# Autodesk Inventor assembly: GI - 100
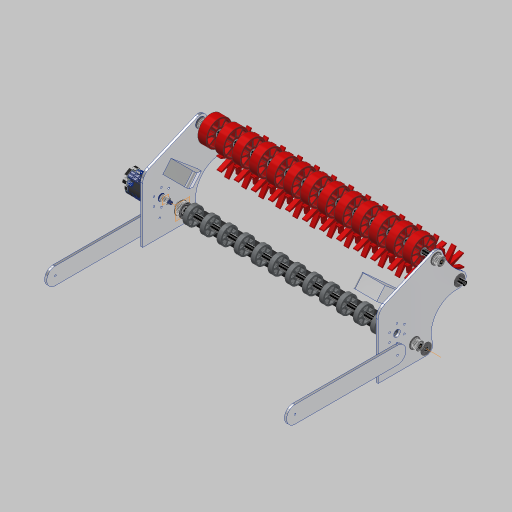
[picture p0: Inventor's stored thumbnail of the model, 512x512]
Saved by Autodesk Inventor 2023.5 (Build 275446000, 446)
## iProperties
Created: 2025-01-18
Part Number: GI - 100
Document SubType Name: Assembly
Designer: mavericks
Author: mavericks
## Documents named in this file (14)
- C:\Users\slick\OneDrive\Desktop\2025-ReefScape---CAD\ground intake\GI - 100.iam
- C:\Users\slick\OneDrive\Desktop\2025-ReefScape---CAD\ground intake\GI - 001.ipt
- C:\Users\slick\OneDrive\Desktop\2025-ReefScape---CAD\COMMON PARTS\BEARINGS\13_75mm_1_2_ThunderHex_ID_x_1_125_OD_x_0_313_WD_Flanged_Bearing_217-4006_MIR.ipt
- C:\Users\slick\OneDrive\Desktop\2025-ReefScape---CAD\ground intake\GI - 002.ipt
- C:\Users\slick\OneDrive\Desktop\2025-ReefScape---CAD\COMMON PARTS\WHEELS\am-0619a .425 Hex Entrapption Star REV2.ipt
- C:\Users\slick\OneDrive\Desktop\2025-ReefScape---CAD\COMMON PARTS\WHEELS\am-3946 3IN 375Hex Compliant Wheel REV 3.ipt
- C:\Users\slick\OneDrive\Desktop\2025-ReefScape---CAD\COMMON PARTS\WHEELS\2_OD_Straight_Flex_Wheel_217-6354.ipt
- C:\Users\slick\OneDrive\Desktop\2025-ReefScape---CAD\ground intake\GI - 200.iam
- C:\Users\slick\OneDrive\Desktop\2025-ReefScape---CAD\COMMON PARTS\MOTORS\Kracken with Cover and Boards.iam
- C:\Users\slick\OneDrive\Desktop\2025-ReefScape---CAD\COMMON PARTS\PULLEYS\gt2\16T Gt2 Kracken PullyWCP-1178.ipt
- C:\Users\slick\OneDrive\Desktop\2025-ReefScape---CAD\COMMON PARTS\PULLEYS\gt2\24t_x_9mm_Wide_Double_Flange_Aluminum_Pulley_GT2_3mm_1_2_Hex_Bore_217-5875.ipt
- C:\Users\slick\OneDrive\Desktop\2025-ReefScape---CAD\COMMON PARTS\PULLEYS\gt2\36t_x_9mm_Wide_Double_Flange_Aluminum_Pulley_GT2_3mm_1_2_Hex_Bore_217-5873.ipt
- C:\Users\slick\OneDrive\Desktop\2025-ReefScape---CAD\ground intake\GI - 005.ipt
- C:\Users\slick\OneDrive\Desktop\2025-ReefScape---CAD\ground intake\GI - 006.ipt
## Components (66 placed, 13 different names)
1. GI - 001:1 — Insert:1, Insert:2, Insert:3, Insert:4, Mate:2, Mate:4, Mate:6, Insert:18, Mate:7, Mate:15, Mate:28, Angle:1, Mate:30, Insert:21
2. 13_75mm_1_2_ThunderHex_ID_x_1_125_OD_x_0_313_WD_Flanged_Bearing_217-4006_MIR:1 — Insert:2, Mate:1, Flush:2, Mate:15, Mate:16, Flush:5, Mate:25, Mate:26
3. 13_75mm_1_2_ThunderHex_ID_x_1_125_OD_x_0_313_WD_Flanged_Bearing_217-4006_MIR:2 — Insert:1, Mate:3, Flush:4, Mate:23, Mate:24
4. 13_75mm_1_2_ThunderHex_ID_x_1_125_OD_x_0_313_WD_Flanged_Bearing_217-4006_MIR:3 — Insert:4, Insert:19
5. 13_75mm_1_2_ThunderHex_ID_x_1_125_OD_x_0_313_WD_Flanged_Bearing_217-4006_MIR:4 — Insert:3, Mate:5, Mate:10, Mate:11, Mate:12, Mate:20, Mate:21
6. GI - 001:2 — Insert:5, Insert:6, Insert:7, Insert:8, Mate:29, Mate:31, Insert:20, Angle:2
7. 13_75mm_1_2_ThunderHex_ID_x_1_125_OD_x_0_313_WD_Flanged_Bearing_217-4006_MIR:5 — Insert:5, Mate:19
8. 13_75mm_1_2_ThunderHex_ID_x_1_125_OD_x_0_313_WD_Flanged_Bearing_217-4006_MIR:6 — Insert:6, Mate:18
9. 13_75mm_1_2_ThunderHex_ID_x_1_125_OD_x_0_313_WD_Flanged_Bearing_217-4006_MIR:7 — Insert:8, Insert:16, Mate:14
10. 13_75mm_1_2_ThunderHex_ID_x_1_125_OD_x_0_313_WD_Flanged_Bearing_217-4006_MIR:8 — Insert:7
11. GI - 002:1 — Mate:18, Flush:4, Mate:27
12. GI - 002:2 — Mate:17, Flush:3, Mate:20, Mate:21
13. GI - 002:4 — Flush:2, Mate:16, Mate:19, Flush:5, Flush:6
14. GI - 200:1 [sub-assembly] — Insert:16, Mate:13, Insert:19
15. Kracken with Cover and Boards:1 [sub-assembly] — Insert:18, Mate:7, Mate:8, Mate:9, Mate:32
16. 16T Gt2 Kracken PullyWCP-1178:1 — Mate:8, Mate:9
17. 24t_x_9mm_Wide_Double_Flange_Aluminum_Pulley_GT2_3mm_1_2_Hex_Bore_217-5875:1 — Mate:10, Flush:1
18. 36t_x_9mm_Wide_Double_Flange_Aluminum_Pulley_GT2_3mm_1_2_Hex_Bore_217-5873:1 — Mate:11, Mate:12
19. 24t_x_9mm_Wide_Double_Flange_Aluminum_Pulley_GT2_3mm_1_2_Hex_Bore_217-5875:2 — Mate:13, Mate:14, Flush:1
20. 24t_x_9mm_Wide_Double_Flange_Aluminum_Pulley_GT2_3mm_1_2_Hex_Bore_217-5875:3 — Mate:17, Flush:3
21. 24t_x_9mm_Wide_Double_Flange_Aluminum_Pulley_GT2_3mm_1_2_Hex_Bore_217-5875:4 — Flush:6, Mate:27
22. 24t_x_9mm_Wide_Double_Flange_Aluminum_Pulley_GT2_3mm_1_2_Hex_Bore_217-5875:5 — Mate:23, Mate:24
23. 24t_x_9mm_Wide_Double_Flange_Aluminum_Pulley_GT2_3mm_1_2_Hex_Bore_217-5875:6 — Mate:25, Mate:26
24. GI - 005:1 — Mate:28, Flush:7, Angle:1, Mate:30, Mate:32
25. GI - 005:2 — Mate:29, Flush:7, Mate:31
26. GI - 006:1 — Insert:20, Angle:2, Flush:8
27. GI - 006:2 — Insert:21, Flush:8
28. am-0619a .425 Hex Entrapption Star REV2:1 — Mate:1, Mate:2
29. am-0619a .425 Hex Entrapption Star REV2:2
30. am-0619a .425 Hex Entrapption Star REV2:3
31. am-0619a .425 Hex Entrapption Star REV2:4
32. am-0619a .425 Hex Entrapption Star REV2:5
33. am-0619a .425 Hex Entrapption Star REV2:6
34. am-0619a .425 Hex Entrapption Star REV2:7
35. am-0619a .425 Hex Entrapption Star REV2:8
36. am-0619a .425 Hex Entrapption Star REV2:9
37. am-0619a .425 Hex Entrapption Star REV2:10
38. am-0619a .425 Hex Entrapption Star REV2:11
39. am-0619a .425 Hex Entrapption Star REV2:12
40. am-0619a .425 Hex Entrapption Star REV2:13
41. am-3946 3IN 375Hex Compliant Wheel REV 3:1 — Mate:3, Mate:4
42. am-3946 3IN 375Hex Compliant Wheel REV 3:2
43. am-3946 3IN 375Hex Compliant Wheel REV 3:3
44. am-3946 3IN 375Hex Compliant Wheel REV 3:4
45. am-3946 3IN 375Hex Compliant Wheel REV 3:5
46. am-3946 3IN 375Hex Compliant Wheel REV 3:6
47. am-3946 3IN 375Hex Compliant Wheel REV 3:7
48. am-3946 3IN 375Hex Compliant Wheel REV 3:8
49. am-3946 3IN 375Hex Compliant Wheel REV 3:9
50. am-3946 3IN 375Hex Compliant Wheel REV 3:10
51. am-3946 3IN 375Hex Compliant Wheel REV 3:11
52. am-3946 3IN 375Hex Compliant Wheel REV 3:12
53. am-3946 3IN 375Hex Compliant Wheel REV 3:13
54. 2_OD_Straight_Flex_Wheel_217-6354:1 — Mate:5, Mate:6
55. 2_OD_Straight_Flex_Wheel_217-6354:2
56. 2_OD_Straight_Flex_Wheel_217-6354:3
57. 2_OD_Straight_Flex_Wheel_217-6354:4
58. 2_OD_Straight_Flex_Wheel_217-6354:5
59. 2_OD_Straight_Flex_Wheel_217-6354:6
60. 2_OD_Straight_Flex_Wheel_217-6354:7
61. 2_OD_Straight_Flex_Wheel_217-6354:8
62. 2_OD_Straight_Flex_Wheel_217-6354:9
63. 2_OD_Straight_Flex_Wheel_217-6354:10
64. 2_OD_Straight_Flex_Wheel_217-6354:11
65. 2_OD_Straight_Flex_Wheel_217-6354:12
66. 2_OD_Straight_Flex_Wheel_217-6354:13
## Component patterns: (13 elements, first: am-0619a .425 Hex Entrapption Star REV2:1), (13 elements, first: am-3946 3IN 375Hex Compliant Wheel REV 3:1), (13 elements, first: 2_OD_Straight_Flex_Wheel_217-6354:1)
## Relationships (54: Mate 31, Insert 13, Flush 8, Angle 2)
- Insert:1: GI - 001:1 ↔ 13_75mm_1_2_ThunderHex_ID_x_1_125_OD_x_0_313_WD_Flanged_Bearing_217-4006_MIR:2
- Insert:2: GI - 001:1 ↔ 13_75mm_1_2_ThunderHex_ID_x_1_125_OD_x_0_313_WD_Flanged_Bearing_217-4006_MIR:1
- Insert:3: GI - 001:1 ↔ 13_75mm_1_2_ThunderHex_ID_x_1_125_OD_x_0_313_WD_Flanged_Bearing_217-4006_MIR:4
- Insert:4: GI - 001:1 ↔ 13_75mm_1_2_ThunderHex_ID_x_1_125_OD_x_0_313_WD_Flanged_Bearing_217-4006_MIR:3
- Insert:5: GI - 001:2 ↔ 13_75mm_1_2_ThunderHex_ID_x_1_125_OD_x_0_313_WD_Flanged_Bearing_217-4006_MIR:5
- Insert:6: GI - 001:2 ↔ 13_75mm_1_2_ThunderHex_ID_x_1_125_OD_x_0_313_WD_Flanged_Bearing_217-4006_MIR:6
- Insert:7: GI - 001:2 ↔ 13_75mm_1_2_ThunderHex_ID_x_1_125_OD_x_0_313_WD_Flanged_Bearing_217-4006_MIR:8
- Insert:8: GI - 001:2 ↔ 13_75mm_1_2_ThunderHex_ID_x_1_125_OD_x_0_313_WD_Flanged_Bearing_217-4006_MIR:7
- Mate:1: 13_75mm_1_2_ThunderHex_ID_x_1_125_OD_x_0_313_WD_Flanged_Bearing_217-4006_MIR:1 ↔ am-0619a .425 Hex Entrapption Star REV2:1
- Mate:2 (36.5125 mm): GI - 001:1 ↔ am-0619a .425 Hex Entrapption Star REV2:1
- Mate:3: 13_75mm_1_2_ThunderHex_ID_x_1_125_OD_x_0_313_WD_Flanged_Bearing_217-4006_MIR:2 ↔ am-3946 3IN 375Hex Compliant Wheel REV 3:1
- Mate:4 (30.1625 mm): GI - 001:1 ↔ am-3946 3IN 375Hex Compliant Wheel REV 3:1
- Mate:5: 13_75mm_1_2_ThunderHex_ID_x_1_125_OD_x_0_313_WD_Flanged_Bearing_217-4006_MIR:4 ↔ 2_OD_Straight_Flex_Wheel_217-6354:1
- Mate:6 (36.5125 mm): GI - 001:1 ↔ 2_OD_Straight_Flex_Wheel_217-6354:1
- Insert:16: 13_75mm_1_2_ThunderHex_ID_x_1_125_OD_x_0_313_WD_Flanged_Bearing_217-4006_MIR:7 ↔ GI - 200:1
- Insert:18: GI - 001:1 ↔ Kracken with Cover and Boards:1
- Mate:7: GI - 001:1 ↔ Kracken with Cover and Boards:1
- Mate:8: Kracken with Cover and Boards:1 ↔ 16T Gt2 Kracken PullyWCP-1178:1
- Mate:9 (3.175 mm): Kracken with Cover and Boards:1 ↔ 16T Gt2 Kracken PullyWCP-1178:1
- Mate:10: 13_75mm_1_2_ThunderHex_ID_x_1_125_OD_x_0_313_WD_Flanged_Bearing_217-4006_MIR:4 ↔ 24t_x_9mm_Wide_Double_Flange_Aluminum_Pulley_GT2_3mm_1_2_Hex_Bore_217-5875:1
- Mate:11: 13_75mm_1_2_ThunderHex_ID_x_1_125_OD_x_0_313_WD_Flanged_Bearing_217-4006_MIR:4 ↔ 36t_x_9mm_Wide_Double_Flange_Aluminum_Pulley_GT2_3mm_1_2_Hex_Bore_217-5873:1
- Mate:12 (3.175 mm): 13_75mm_1_2_ThunderHex_ID_x_1_125_OD_x_0_313_WD_Flanged_Bearing_217-4006_MIR:4 ↔ 36t_x_9mm_Wide_Double_Flange_Aluminum_Pulley_GT2_3mm_1_2_Hex_Bore_217-5873:1
- Mate:13: GI - 200:1 ↔ 24t_x_9mm_Wide_Double_Flange_Aluminum_Pulley_GT2_3mm_1_2_Hex_Bore_217-5875:2
- Mate:14: 13_75mm_1_2_ThunderHex_ID_x_1_125_OD_x_0_313_WD_Flanged_Bearing_217-4006_MIR:7 ↔ 24t_x_9mm_Wide_Double_Flange_Aluminum_Pulley_GT2_3mm_1_2_Hex_Bore_217-5875:2
- Flush:1: 24t_x_9mm_Wide_Double_Flange_Aluminum_Pulley_GT2_3mm_1_2_Hex_Bore_217-5875:1 ↔ 24t_x_9mm_Wide_Double_Flange_Aluminum_Pulley_GT2_3mm_1_2_Hex_Bore_217-5875:2
- Flush:2: 13_75mm_1_2_ThunderHex_ID_x_1_125_OD_x_0_313_WD_Flanged_Bearing_217-4006_MIR:1 ↔ GI - 002:4
- Mate:15: GI - 001:1 ↔ 13_75mm_1_2_ThunderHex_ID_x_1_125_OD_x_0_313_WD_Flanged_Bearing_217-4006_MIR:1
- Mate:16: 13_75mm_1_2_ThunderHex_ID_x_1_125_OD_x_0_313_WD_Flanged_Bearing_217-4006_MIR:1 ↔ GI - 002:4
- Insert:19: 13_75mm_1_2_ThunderHex_ID_x_1_125_OD_x_0_313_WD_Flanged_Bearing_217-4006_MIR:3 ↔ GI - 200:1
- Mate:17: GI - 002:2 ↔ 24t_x_9mm_Wide_Double_Flange_Aluminum_Pulley_GT2_3mm_1_2_Hex_Bore_217-5875:3
- Flush:3: GI - 002:2 ↔ 24t_x_9mm_Wide_Double_Flange_Aluminum_Pulley_GT2_3mm_1_2_Hex_Bore_217-5875:3
- Mate:18: 13_75mm_1_2_ThunderHex_ID_x_1_125_OD_x_0_313_WD_Flanged_Bearing_217-4006_MIR:6 ↔ GI - 002:1
- Mate:19: 13_75mm_1_2_ThunderHex_ID_x_1_125_OD_x_0_313_WD_Flanged_Bearing_217-4006_MIR:5 ↔ GI - 002:4
- Flush:4: 13_75mm_1_2_ThunderHex_ID_x_1_125_OD_x_0_313_WD_Flanged_Bearing_217-4006_MIR:2 ↔ GI - 002:1
- Flush:5: 13_75mm_1_2_ThunderHex_ID_x_1_125_OD_x_0_313_WD_Flanged_Bearing_217-4006_MIR:1 ↔ GI - 002:4
- Mate:20: 13_75mm_1_2_ThunderHex_ID_x_1_125_OD_x_0_313_WD_Flanged_Bearing_217-4006_MIR:4 ↔ GI - 002:2
- Mate:21: 13_75mm_1_2_ThunderHex_ID_x_1_125_OD_x_0_313_WD_Flanged_Bearing_217-4006_MIR:4 ↔ GI - 002:2
- Flush:6: GI - 002:4 ↔ 24t_x_9mm_Wide_Double_Flange_Aluminum_Pulley_GT2_3mm_1_2_Hex_Bore_217-5875:4
- Mate:23: 13_75mm_1_2_ThunderHex_ID_x_1_125_OD_x_0_313_WD_Flanged_Bearing_217-4006_MIR:2 ↔ 24t_x_9mm_Wide_Double_Flange_Aluminum_Pulley_GT2_3mm_1_2_Hex_Bore_217-5875:5
- Mate:24 (3.175 mm): 13_75mm_1_2_ThunderHex_ID_x_1_125_OD_x_0_313_WD_Flanged_Bearing_217-4006_MIR:2 ↔ 24t_x_9mm_Wide_Double_Flange_Aluminum_Pulley_GT2_3mm_1_2_Hex_Bore_217-5875:5
- Mate:25: 13_75mm_1_2_ThunderHex_ID_x_1_125_OD_x_0_313_WD_Flanged_Bearing_217-4006_MIR:1 ↔ 24t_x_9mm_Wide_Double_Flange_Aluminum_Pulley_GT2_3mm_1_2_Hex_Bore_217-5875:6
- Mate:26 (3.175 mm): 13_75mm_1_2_ThunderHex_ID_x_1_125_OD_x_0_313_WD_Flanged_Bearing_217-4006_MIR:1 ↔ 24t_x_9mm_Wide_Double_Flange_Aluminum_Pulley_GT2_3mm_1_2_Hex_Bore_217-5875:6
- Mate:27: GI - 002:1 ↔ 24t_x_9mm_Wide_Double_Flange_Aluminum_Pulley_GT2_3mm_1_2_Hex_Bore_217-5875:4
- Mate:28: GI - 001:1 ↔ GI - 005:1
- Mate:29: GI - 001:2 ↔ GI - 005:2
- Flush:7: GI - 005:1 ↔ GI - 005:2
- Angle:1 (40 deg): GI - 001:1 ↔ GI - 005:1
- Mate:30 (101.6 mm): GI - 001:1 ↔ GI - 005:1
- Mate:31 (177.8 mm): GI - 001:2 ↔ GI - 005:2
- Mate:32 (57.15 mm): Kracken with Cover and Boards:1 ↔ GI - 005:1
- Insert:20: GI - 001:2 ↔ GI - 006:1
- Insert:21: GI - 001:1 ↔ GI - 006:2
- Angle:2 (0 deg): GI - 001:2 ↔ GI - 006:1
- Flush:8: GI - 006:1 ↔ GI - 006:2
